# Autodesk Inventor assembly: Body
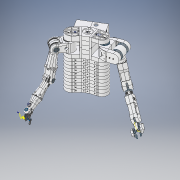
[picture p0: Inventor's stored thumbnail of the model, 180x180]
Saved by Autodesk Inventor 2017 SP1 (Build 210196100, 196)
## iProperties
Created: 2017-03-13
Part Number: Body
Document SubType Name: Assembly
Designer: zallen
Author: zallen
## Documents named in this file (3)
- C:\Users\Zach\Documents\GitHub\tr1\src\Body\Body.iam
- C:\Users\Zach\Documents\GitHub\tr1\src\Body\Chest Assembly\Chest Assembly.iam
- C:\Users\Zach\Documents\GitHub\tr1\src\Body\Arm 2.0 Assembly\Arm 2.0 Assembly.iam
## Components (3 placed, 2 different names)
1. Chest Assembly:1 [sub-assembly] — Mate:3, Mate:4, Mate:5, Mate:6, Mate:7, Mate:8
2. Arm 2.0 Assembly:1 [sub-assembly] — Mate:3, Mate:4
3. Arm 2.0 Assembly:2 [sub-assembly] — Mate:5, Mate:6, Mate:7, Mate:8
## Relationships (6: Mate 6)
- Mate:3: Chest Assembly:1 ↔ Arm 2.0 Assembly:1
- Mate:4: Chest Assembly:1 ↔ Arm 2.0 Assembly:1
- Mate:5: Chest Assembly:1 ↔ Arm 2.0 Assembly:2
- Mate:6: Chest Assembly:1 ↔ Arm 2.0 Assembly:2
- Mate:7: Chest Assembly:1 ↔ Arm 2.0 Assembly:2
- Mate:8: Chest Assembly:1 ↔ Arm 2.0 Assembly:2
